# Autodesk Inventor assembly: The-Compleat-Thing
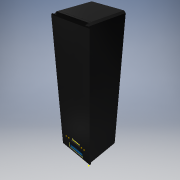
[picture p0: Inventor's stored thumbnail of the model, 180x180]
Saved by Autodesk Inventor 2019 (Build 230136000, 136)
## iProperties
Created: 2018-12-05
Part Number: The-Compleat-Thing
Document SubType Name: Assembly
Designer: lateSWE
Author: lateSWE
## Documents named in this file (5)
- C:\Users\lateSWE\Documents\Inventor\Modular Power-Bank\The-Compleat-Thing.iam
- C:\Users\lateSWE\Documents\Inventor\Modular Power-Bank\18650-battery.ipt
- C:\Users\lateSWE\Documents\Inventor\Modular Power-Bank\Battery-Management.ipt
- C:\Users\lateSWE\Documents\Inventor\Modular Power-Bank\1-Battery-Management-Case.ipt
- C:\Users\lateSWE\Documents\Inventor\Modular Power-Bank\Battery-Management-Case-Cover.ipt
## Components (4 placed, 4 different names)
1. 18650-battery:1 — Rigid:1
2. Battery-Management:1 — Rigid:2
3. 1-Battery-Management-Case:1 — Rigid:1, Rigid:2, Rigid:3
4. Battery-Management-Case-Cover:1 — Rigid:3
## Relationships (3: WeldJoint 3)
- Rigid:1 [WeldJoint] (0.5 mm): 18650-battery:1 ↔ 1-Battery-Management-Case:1
- Rigid:2 [WeldJoint] (2.25 mm): Battery-Management:1 ↔ 1-Battery-Management-Case:1
- Rigid:3 [WeldJoint]: 1-Battery-Management-Case:1 ↔ Battery-Management-Case-Cover:1
